# Autodesk Inventor assembly: y_carryage
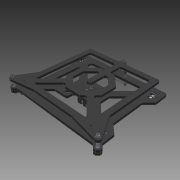
[picture p0: Inventor's stored thumbnail of the model, 180x180]
Saved by Autodesk Inventor 2014 (Build 180170000, 170)
## iProperties
Created: 2014-04-02
Part Number: y_carryage
Document SubType Name: Assembly
Designer: buben
Author: buben
## Documents named in this file (17)
- C:\Users\buben\Documents\GitHub\bacon\inventor files\assemblies\y_carryage.iam
- C:\Users\buben\Documents\GitHub\bacon\inventor files\printer parts\y_carriage.ipt
- C:\Users\buben\Documents\GitHub\bacon\inventor files\3rd party components\linear_bearing_8\Imported Components\LU8MM\LU8MM.iam
- C:\Users\buben\Documents\GitHub\bacon\inventor files\utils\y_carryage_bearing_zip_tie.ipt
- C:\Users\buben\Documents\GitHub\bacon\inventor files\printer parts\y_carriage_belt_mount.ipt
- C:\Users\buben\Documents\GitHub\bacon\inventor files\printer parts\y_carriage_belt_mount_bed_holder.ipt
- C:\Users\buben\Documents\GitHub\bacon\inventor files\utils\washer_m4.ipt
- C:\Users\buben\Documents\Inventor\Content Center Files\R2014\en-US\ISO 7040\ISO 7040 - M4.ipt
- C:\Users\buben\Documents\Inventor\Content Center Files\R2014\en-US\ISO 4762(2)\ISO 4762 - M4 x 30ISO.ipt
- C:\Users\buben\Documents\GitHub\bacon\inventor files\utils\washer_m5.ipt
- C:\Users\buben\Documents\GitHub\bacon\inventor files\printer parts\y_carriage_nut_holder_a.ipt
- C:\Users\buben\Documents\Inventor\Content Center Files\R2014\en-US\ISO 4762(2)\ISO 4762 - M4 x 25ISO.ipt
- C:\Users\buben\Documents\GitHub\bacon\inventor files\printer parts\y_carriage_nut_holder_b.ipt
- C:\Users\buben\Documents\GitHub\bacon\inventor files\utils\y_carryage_spring.ipt
- C:\Users\buben\Documents\GitHub\bacon\inventor files\printer parts\heatbed_mount.ipt
- C:\Users\buben\Documents\Inventor\Content Center Files\R2014\en-US\CSN EN 24032\ISO 4032 - M5CSN EN.ipt
- C:\Users\buben\Documents\Inventor\Content Center Files\R2014\en-US\ISO 4762(2)\ISO 4762 - M5 x 45ISO.ipt
## Components (77 placed, 16 different names)
1. y_carriage:1 — Mate:1, Mate:2, Mate:3, Mate:4, Mate:5, Mate:6, Mate:7, Mate:8, Mate:9, Mate:12, Mate:13, Angle:1, Angle:2, Angle:3, Angle:4, Angle:5, Angle:6, Angle:7, Angle:8, Mate:22, Mate:23, Mate:24, Mate:25, Mate:26, Mate:27, Mate:28, Mate:29, Mate:36, Mate:37, Mate:38, Mate:39, Mate:40, Mate:41, Mate:42, Mate:63, Mate:64, Mate:65, Mate:66, Mate:67, Mate:68, Mate:69, Mate:70, Mate:71, Mate:72, Mate:74, Mate:76, Angle:9, Angle:10, Mate:81, Mate:82, Mate:83, Mate:84, Mate:89, Mate:90, Mate:91, Mate:92, Mate:94, Mate:95, Mate:98, Mate:99, Mate:100, Mate:101, Mate:108, Mate:109, Mate:110, Mate:111, Mate:112, Mate:113, Mate:121, Mate:123, Mate:125, Mate:127, Mate:144
2. LU8MM:1 [sub-assembly] — Mate:4, Mate:5, Mate:9, Mate:10, Mate:16, Mate:17
3. LU8MM:2 [sub-assembly] — Mate:6, Mate:7, Mate:8, Mate:11, Mate:14, Mate:15
4. LU8MM:3 [sub-assembly] — Mate:10, Mate:12, Mate:18, Mate:19
5. LU8MM:4 [sub-assembly] — Mate:11, Mate:13, Mate:20, Mate:21
6. y_carryage_bearing_zip_tie:1 — Mate:19, Angle:7, Mate:22
7. y_carryage_bearing_zip_tie:2 — Mate:17, Angle:5, Mate:28
8. y_carryage_bearing_zip_tie:3 — Mate:15, Angle:2, Mate:27
9. y_carryage_bearing_zip_tie:4 — Mate:14, Angle:1, Mate:26
10. y_carryage_bearing_zip_tie:5 — Mate:21, Angle:3, Mate:25
11. y_carryage_bearing_zip_tie:6 — Mate:20, Angle:4, Mate:24
12. y_carryage_bearing_zip_tie:7 — Mate:18, Angle:8, Mate:23
13. y_carryage_bearing_zip_tie:8 — Mate:16, Angle:6, Mate:29
14. y_carriage_belt_mount:1 — Mate:31, Mate:34, Mate:35, Mate:36, Mate:37, Mate:51, Mate:52, Mate:55, Mate:56
15. y_carriage_belt_mount:2 — Mate:30, Mate:32, Mate:33, Mate:38, Mate:53, Mate:54
16. y_carriage_belt_mount_bed_holder:1 — Mate:30, Mate:31, Mate:32, Mate:33, Mate:34, Mate:35, Mate:43, Mate:44
17. CSN 02 1702 B B 4,3:1 — Mate:40, Mate:41, Insert:1
18. CSN 02 1702 B B 4,3:2 — Mate:43, Mate:46, Mate:49
19. CSN 02 1702 B B 4,3:3 — Mate:44, Mate:45, Mate:47
20. CSN 02 1702 B B 4,3:4 — Mate:39, Mate:42, Insert:2
21. ISO 4762 M4 x 30:1 — Insert:1, Mate:45, Mate:48
22. ISO 4762 M4 x 30:2 — Insert:2, Mate:46, Mate:50
23. DIN EN ISO 7040 M4:1 — Mate:47, Mate:48
24. DIN EN ISO 7040 M4:2 — Mate:49, Mate:50
25. CSN 02 1702 B B 4,3:5 — Mate:51, Mate:55, Insert:4
26. CSN 02 1702 B B 4,3:6 — Mate:52, Mate:56, Insert:3
27. CSN 02 1702 B B 4,3:7 — Mate:54, Mate:58, Mate:61
28. CSN 02 1702 B B 4,3:8 — Mate:53, Mate:57, Mate:59
29. ISO 4762 M4 x 30:4 — Insert:3, Mate:57, Mate:60
30. ISO 4762 M4 x 30:3 — Insert:4, Mate:58, Mate:62
31. DIN EN ISO 7040 M4:3 — Mate:61, Mate:62
32. DIN EN ISO 7040 M4:4 — Mate:59, Mate:60
33. CSN 02 1702 B B 5,3:1 — Mate:71, Mate:72, Mate:93, Mate:141
34. CSN 02 1702 B B 5,3:2 — Mate:68, Mate:69, Mate:75, Mate:135
35. CSN 02 1702 B B 5,3:3 — Mate:65, Mate:66, Mate:73, Mate:138
36. CSN 02 1702 B B 4,3:9 — Mate:64, Mate:70
37. CSN 02 1702 B B 4,3:10 — Mate:63, Mate:67
38. CSN 02 1702 B B 4,3:11 — Mate:79, Mate:80, Mate:85
39. CSN 02 1702 B B 4,3:12 — Mate:77, Mate:78, Mate:87
40. y_carriage_nut_holder_a:1 — Mate:73, Mate:74, Angle:10, Mate:77, Mate:78, Mate:139, Mate:140
41. y_carriage_nut_holder_a:2 — Mate:75, Mate:76, Angle:9, Mate:79, Mate:80, Mate:136, Mate:137
42. CSN 02 1702 B B 4,3:13 — Mate:83, Mate:84, Insert:5
43. CSN 02 1702 B B 4,3:14 — Mate:81, Mate:82, Insert:6
44. ISO 4762 M4 x 25:2 — Insert:5, Mate:86
45. ISO 4762 M4 x 25:1 — Insert:6, Mate:88
46. DIN EN ISO 7040 M4:5 — Mate:85, Mate:86
47. DIN EN ISO 7040 M4:6 — Mate:87, Mate:88
48. CSN 02 1702 B B 4,3:15 — Mate:90, Mate:91
49. CSN 02 1702 B B 4,3:16 — Mate:89, Mate:92
50. y_carriage_nut_holder_b:1 — Mate:93, Mate:94, Mate:95, Mate:96, Mate:97, Mate:142, Mate:143
51. CSN 02 1702 B B 4,3:17 — Mate:96, Mate:103, Mate:104
52. CSN 02 1702 B B 4,3:18 — Mate:97, Mate:102, Mate:106
53. CSN 02 1702 B B 4,3:19 — Mate:98, Mate:101, Insert:7
54. CSN 02 1702 B B 4,3:20 — Mate:99, Mate:100, Insert:8
55. ISO 4762 M4 x 25:3 — Insert:7, Mate:102, Mate:107
56. ISO 4762 M4 x 25:4 — Insert:8, Mate:103, Mate:105
57. DIN EN ISO 7040 M4:7 — Mate:106, Mate:107
58. DIN EN ISO 7040 M4:8 — Mate:104, Mate:105
59. CSN 02 1702 B B 5,3:4 — Mate:110, Mate:111, Mate:115, Mate:118
60. CSN 02 1702 B B 5,3:5 — Mate:108, Mate:112, Mate:116, Mate:119
61. CSN 02 1702 B B 5,3:6 — Mate:109, Mate:113, Mate:114, Mate:117
62. CSN 02 1702 B B 5,3:7 — Mate:124, Mate:125
63. CSN 02 1702 B B 5,3:8 — Mate:122, Mate:123
64. CSN 02 1702 B B 5,3:9 — Mate:120, Mate:121, Mate:126
65. CSN 02 1702 B B 5,3:10 — Mate:129, Mate:133, Insert:10
66. CSN 02 1702 B B 5,3:11 — Mate:130, Mate:132, Insert:11
67. CSN 02 1702 B B 5,3:12 — Mate:131, Mate:134, Insert:9
68. Compress Spring1:1 — Mate:114, Mate:117, Mate:124
69. Compress Spring1:2 — Mate:115, Mate:118, Mate:122
70. Compress Spring1:3 — Mate:116, Mate:119, Mate:120
71. heatbed_mount:1 — Mate:126, Mate:127, Mate:129, Mate:130, Mate:131, Mate:132, Mate:133, Mate:134, Mate:144
72. CSN EN 24032 M5:1 — Mate:135, Mate:136, Mate:137
73. CSN EN 24032 M5:2 — Mate:141, Mate:142, Mate:143
74. CSN EN 24032 M5:3 — Mate:138, Mate:139, Mate:140
75. ISO 4762 M5 x 45:2 — Insert:9
76. ISO 4762 M5 x 45:3 — Insert:10
77. ISO 4762 M5 x 45:1 — Insert:11
## Relationships (164: Mate 143, Insert 11, Angle 10)
- Mate:1: y_carriage:1
- Mate:2: y_carriage:1
- Mate:3: y_carriage:1
- Mate:4 (7.5 mm): y_carriage:1 ↔ LU8MM:1
- Mate:5 (7.5 mm): y_carriage:1 ↔ LU8MM:1
- Mate:6 (7.5 mm): y_carriage:1 ↔ LU8MM:2
- Mate:7 (7.5 mm): y_carriage:1 ↔ LU8MM:2
- Mate:8 (0.5 mm): y_carriage:1 ↔ LU8MM:2
- Mate:9 (0.5 mm): y_carriage:1 ↔ LU8MM:1
- Mate:10: LU8MM:1 ↔ LU8MM:3
- Mate:11: LU8MM:2 ↔ LU8MM:4
- Mate:12 (0.5 mm): y_carriage:1 ↔ LU8MM:3
- Mate:13 (0.5 mm): y_carriage:1 ↔ LU8MM:4
- Mate:14: LU8MM:2 ↔ y_carryage_bearing_zip_tie:4
- Mate:15: LU8MM:2 ↔ y_carryage_bearing_zip_tie:3
- Mate:16: LU8MM:1 ↔ y_carryage_bearing_zip_tie:8
- Mate:17: LU8MM:1 ↔ y_carryage_bearing_zip_tie:2
- Mate:18: LU8MM:3 ↔ y_carryage_bearing_zip_tie:7
- Mate:19: LU8MM:3 ↔ y_carryage_bearing_zip_tie:1
- Mate:20: LU8MM:4 ↔ y_carryage_bearing_zip_tie:6
- Mate:21: LU8MM:4 ↔ y_carryage_bearing_zip_tie:5
- Angle:1 (180 deg): y_carriage:1 ↔ y_carryage_bearing_zip_tie:4
- Angle:2 (180 deg): y_carriage:1 ↔ y_carryage_bearing_zip_tie:3
- Angle:3 (180 deg): y_carriage:1 ↔ y_carryage_bearing_zip_tie:5
- Angle:4 (180 deg): y_carriage:1 ↔ y_carryage_bearing_zip_tie:6
- Angle:5 (180 deg): y_carriage:1 ↔ y_carryage_bearing_zip_tie:2
- Angle:6 (180 deg): y_carriage:1 ↔ y_carryage_bearing_zip_tie:8
- Angle:7 (180 deg): y_carriage:1 ↔ y_carryage_bearing_zip_tie:1
- Angle:8 (180 deg): y_carriage:1 ↔ y_carryage_bearing_zip_tie:7
- Mate:22 (5 mm): y_carriage:1 ↔ y_carryage_bearing_zip_tie:1
- Mate:23 (5 mm): y_carriage:1 ↔ y_carryage_bearing_zip_tie:7
- Mate:24 (5 mm): y_carriage:1 ↔ y_carryage_bearing_zip_tie:6
- Mate:25 (5 mm): y_carriage:1 ↔ y_carryage_bearing_zip_tie:5
- Mate:26 (5 mm): y_carriage:1 ↔ y_carryage_bearing_zip_tie:4
- Mate:27 (5 mm): y_carriage:1 ↔ y_carryage_bearing_zip_tie:3
- Mate:28 (5 mm): y_carriage:1 ↔ y_carryage_bearing_zip_tie:2
- Mate:29 (5 mm): y_carriage:1 ↔ y_carryage_bearing_zip_tie:8
- Mate:30: y_carriage_belt_mount:2 ↔ y_carriage_belt_mount_bed_holder:1
- Mate:31: y_carriage_belt_mount:1 ↔ y_carriage_belt_mount_bed_holder:1
- Mate:32: y_carriage_belt_mount:2 ↔ y_carriage_belt_mount_bed_holder:1
- Mate:33: y_carriage_belt_mount:2 ↔ y_carriage_belt_mount_bed_holder:1
- Mate:34: y_carriage_belt_mount:1 ↔ y_carriage_belt_mount_bed_holder:1
- Mate:35: y_carriage_belt_mount:1 ↔ y_carriage_belt_mount_bed_holder:1
- Mate:36: y_carriage:1 ↔ y_carriage_belt_mount:1
- Mate:37: y_carriage:1 ↔ y_carriage_belt_mount:1
- Mate:38: y_carriage:1 ↔ y_carriage_belt_mount:2
- Mate:39: y_carriage:1 ↔ CSN 02 1702 B B 4,3:4
- Mate:40: y_carriage:1 ↔ CSN 02 1702 B B 4,3:1
- Mate:41: y_carriage:1 ↔ CSN 02 1702 B B 4,3:1
- Mate:42: y_carriage:1 ↔ CSN 02 1702 B B 4,3:4
- Insert:1: CSN 02 1702 B B 4,3:1 ↔ ISO 4762 M4 x 30:1
- Insert:2: CSN 02 1702 B B 4,3:4 ↔ ISO 4762 M4 x 30:2
- Mate:43: y_carriage_belt_mount_bed_holder:1 ↔ CSN 02 1702 B B 4,3:2
- Mate:44: y_carriage_belt_mount_bed_holder:1 ↔ CSN 02 1702 B B 4,3:3
- Mate:45: CSN 02 1702 B B 4,3:3 ↔ ISO 4762 M4 x 30:1
- Mate:46: CSN 02 1702 B B 4,3:2 ↔ ISO 4762 M4 x 30:2
- Mate:47: CSN 02 1702 B B 4,3:3 ↔ DIN EN ISO 7040 M4:1
- Mate:48: ISO 4762 M4 x 30:1 ↔ DIN EN ISO 7040 M4:1
- Mate:49: CSN 02 1702 B B 4,3:2 ↔ DIN EN ISO 7040 M4:2
- Mate:50: ISO 4762 M4 x 30:2 ↔ DIN EN ISO 7040 M4:2
- Mate:51: y_carriage_belt_mount:1 ↔ CSN 02 1702 B B 4,3:5
- Mate:52: y_carriage_belt_mount:1 ↔ CSN 02 1702 B B 4,3:6
- Mate:53: y_carriage_belt_mount:2 ↔ CSN 02 1702 B B 4,3:8
- Mate:54: y_carriage_belt_mount:2 ↔ CSN 02 1702 B B 4,3:7
- Mate:55: y_carriage_belt_mount:1 ↔ CSN 02 1702 B B 4,3:5
- Mate:56: y_carriage_belt_mount:1 ↔ CSN 02 1702 B B 4,3:6
- Insert:3: CSN 02 1702 B B 4,3:6 ↔ ISO 4762 M4 x 30:4
- Insert:4: CSN 02 1702 B B 4,3:5 ↔ ISO 4762 M4 x 30:3
- Mate:57: CSN 02 1702 B B 4,3:8 ↔ ISO 4762 M4 x 30:4
- Mate:58: CSN 02 1702 B B 4,3:7 ↔ ISO 4762 M4 x 30:3
- Mate:59: CSN 02 1702 B B 4,3:8 ↔ DIN EN ISO 7040 M4:4
- Mate:60: ISO 4762 M4 x 30:4 ↔ DIN EN ISO 7040 M4:4
- Mate:61: CSN 02 1702 B B 4,3:7 ↔ DIN EN ISO 7040 M4:3
- Mate:62: ISO 4762 M4 x 30:3 ↔ DIN EN ISO 7040 M4:3
- Mate:63: y_carriage:1 ↔ CSN 02 1702 B B 4,3:10
- Mate:64: y_carriage:1 ↔ CSN 02 1702 B B 4,3:9
- Mate:65: y_carriage:1 ↔ CSN 02 1702 B B 5,3:3
- Mate:66: y_carriage:1 ↔ CSN 02 1702 B B 5,3:3
- Mate:67: y_carriage:1 ↔ CSN 02 1702 B B 4,3:10
- Mate:68: y_carriage:1 ↔ CSN 02 1702 B B 5,3:2
- Mate:69: y_carriage:1 ↔ CSN 02 1702 B B 5,3:2
- Mate:70: y_carriage:1 ↔ CSN 02 1702 B B 4,3:9
- Mate:71: y_carriage:1 ↔ CSN 02 1702 B B 5,3:1
- Mate:72: y_carriage:1 ↔ CSN 02 1702 B B 5,3:1
- Mate:73: CSN 02 1702 B B 5,3:3 ↔ y_carriage_nut_holder_a:1
- Mate:74: y_carriage:1 ↔ y_carriage_nut_holder_a:1
- Mate:75: CSN 02 1702 B B 5,3:2 ↔ y_carriage_nut_holder_a:2
- Mate:76: y_carriage:1 ↔ y_carriage_nut_holder_a:2
- Angle:9 (0 deg): y_carriage:1 ↔ y_carriage_nut_holder_a:2
- Angle:10 (0 deg): y_carriage:1 ↔ y_carriage_nut_holder_a:1
- Mate:77: CSN 02 1702 B B 4,3:12 ↔ y_carriage_nut_holder_a:1
- Mate:78: CSN 02 1702 B B 4,3:12 ↔ y_carriage_nut_holder_a:1
- Mate:79: CSN 02 1702 B B 4,3:11 ↔ y_carriage_nut_holder_a:2
- Mate:80: CSN 02 1702 B B 4,3:11 ↔ y_carriage_nut_holder_a:2
- Mate:81: y_carriage:1 ↔ CSN 02 1702 B B 4,3:14
- Mate:82: y_carriage:1 ↔ CSN 02 1702 B B 4,3:14
- Mate:83: y_carriage:1 ↔ CSN 02 1702 B B 4,3:13
- Mate:84: y_carriage:1 ↔ CSN 02 1702 B B 4,3:13
- Insert:5: CSN 02 1702 B B 4,3:13 ↔ ISO 4762 M4 x 25:2
- Insert:6: CSN 02 1702 B B 4,3:14 ↔ ISO 4762 M4 x 25:1
- Mate:85: CSN 02 1702 B B 4,3:11 ↔ DIN EN ISO 7040 M4:5
- Mate:86: ISO 4762 M4 x 25:2 ↔ DIN EN ISO 7040 M4:5
- Mate:87: CSN 02 1702 B B 4,3:12 ↔ DIN EN ISO 7040 M4:6
- Mate:88: ISO 4762 M4 x 25:1 ↔ DIN EN ISO 7040 M4:6
- Mate:89: y_carriage:1 ↔ CSN 02 1702 B B 4,3:16
- Mate:90: y_carriage:1 ↔ CSN 02 1702 B B 4,3:15
- Mate:91: y_carriage:1 ↔ CSN 02 1702 B B 4,3:15
- Mate:92: y_carriage:1 ↔ CSN 02 1702 B B 4,3:16
- Mate:93: CSN 02 1702 B B 5,3:1 ↔ y_carriage_nut_holder_b:1
- Mate:94: y_carriage:1 ↔ y_carriage_nut_holder_b:1
- Mate:95: y_carriage:1 ↔ y_carriage_nut_holder_b:1
- Mate:96: y_carriage_nut_holder_b:1 ↔ CSN 02 1702 B B 4,3:17
- Mate:97: y_carriage_nut_holder_b:1 ↔ CSN 02 1702 B B 4,3:18
- Mate:98: y_carriage:1 ↔ CSN 02 1702 B B 4,3:19
- Mate:99: y_carriage:1 ↔ CSN 02 1702 B B 4,3:20
- Mate:100: y_carriage:1 ↔ CSN 02 1702 B B 4,3:20
- Mate:101: y_carriage:1 ↔ CSN 02 1702 B B 4,3:19
- Insert:7: CSN 02 1702 B B 4,3:19 ↔ ISO 4762 M4 x 25:3
- Insert:8: CSN 02 1702 B B 4,3:20 ↔ ISO 4762 M4 x 25:4
- Mate:102: CSN 02 1702 B B 4,3:18 ↔ ISO 4762 M4 x 25:3
- Mate:103: CSN 02 1702 B B 4,3:17 ↔ ISO 4762 M4 x 25:4
- Mate:104: CSN 02 1702 B B 4,3:17 ↔ DIN EN ISO 7040 M4:8
- Mate:105: ISO 4762 M4 x 25:4 ↔ DIN EN ISO 7040 M4:8
- Mate:106: CSN 02 1702 B B 4,3:18 ↔ DIN EN ISO 7040 M4:7
- Mate:107: ISO 4762 M4 x 25:3 ↔ DIN EN ISO 7040 M4:7
- Mate:108: y_carriage:1 ↔ CSN 02 1702 B B 5,3:5
- Mate:109: y_carriage:1 ↔ CSN 02 1702 B B 5,3:6
- Mate:110: y_carriage:1 ↔ CSN 02 1702 B B 5,3:4
- Mate:111: y_carriage:1 ↔ CSN 02 1702 B B 5,3:4
- Mate:112: y_carriage:1 ↔ CSN 02 1702 B B 5,3:5
- Mate:113: y_carriage:1 ↔ CSN 02 1702 B B 5,3:6
- Mate:114: CSN 02 1702 B B 5,3:6 ↔ Compress Spring1:1
- Mate:115: CSN 02 1702 B B 5,3:4 ↔ Compress Spring1:2
- Mate:116: CSN 02 1702 B B 5,3:5 ↔ Compress Spring1:3
- Mate:117: CSN 02 1702 B B 5,3:6 ↔ Compress Spring1:1
- Mate:118: CSN 02 1702 B B 5,3:4 ↔ Compress Spring1:2
- Mate:119: CSN 02 1702 B B 5,3:5 ↔ Compress Spring1:3
- Mate:120: CSN 02 1702 B B 5,3:9 ↔ Compress Spring1:3
- Mate:121: y_carriage:1 ↔ CSN 02 1702 B B 5,3:9
- Mate:122: CSN 02 1702 B B 5,3:8 ↔ Compress Spring1:2
- Mate:123: y_carriage:1 ↔ CSN 02 1702 B B 5,3:8
- Mate:124: CSN 02 1702 B B 5,3:7 ↔ Compress Spring1:1
- Mate:125: y_carriage:1 ↔ CSN 02 1702 B B 5,3:7
- Mate:126: CSN 02 1702 B B 5,3:9 ↔ heatbed_mount:1
- Mate:127: y_carriage:1 ↔ heatbed_mount:1
- Mate:129: CSN 02 1702 B B 5,3:10 ↔ heatbed_mount:1
- Mate:130: CSN 02 1702 B B 5,3:11 ↔ heatbed_mount:1
- Mate:131: CSN 02 1702 B B 5,3:12 ↔ heatbed_mount:1
- Mate:132: CSN 02 1702 B B 5,3:11 ↔ heatbed_mount:1
- Mate:133: CSN 02 1702 B B 5,3:10 ↔ heatbed_mount:1
- Mate:134: CSN 02 1702 B B 5,3:12 ↔ heatbed_mount:1
- Mate:135: CSN 02 1702 B B 5,3:2 ↔ CSN EN 24032 M5:1
- Mate:136: y_carriage_nut_holder_a:2 ↔ CSN EN 24032 M5:1
- Mate:137: y_carriage_nut_holder_a:2 ↔ CSN EN 24032 M5:1
- Mate:138: CSN 02 1702 B B 5,3:3 ↔ CSN EN 24032 M5:3
- Mate:139: y_carriage_nut_holder_a:1 ↔ CSN EN 24032 M5:3
- Mate:140: y_carriage_nut_holder_a:1 ↔ CSN EN 24032 M5:3
- Mate:141: CSN 02 1702 B B 5,3:1 ↔ CSN EN 24032 M5:2
- Mate:142: y_carriage_nut_holder_b:1 ↔ CSN EN 24032 M5:2
- Mate:143: y_carriage_nut_holder_b:1 ↔ CSN EN 24032 M5:2
- Mate:144: y_carriage:1 ↔ heatbed_mount:1
- Insert:9: CSN 02 1702 B B 5,3:12 ↔ ISO 4762 M5 x 45:2
- Insert:10: CSN 02 1702 B B 5,3:10 ↔ ISO 4762 M5 x 45:3
- Insert:11: CSN 02 1702 B B 5,3:11 ↔ ISO 4762 M5 x 45:1
